# Autodesk Inventor assembly: КВ33.044.500 - Каретка оси Y
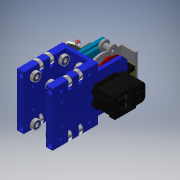
[picture p0: Inventor's stored thumbnail of the model, 180x180]
Saved by Autodesk Inventor 2019 (Build 230136000, 136)
## iProperties
Created: 2019-07-21
Part Number: КВ33.044.500 - Каретка оси Y
Material: Типовые
Document SubType Name: Assembly
Designer: Петров Иван
Mass: 285.838 g
Surface Area: 1117.75 cm^2
Volume: 225.546 cm^3
Density: 1.26732 g/cm^3
Author: Петров Иван
## Documents named in this file (14)
- E:\IVAN\Kvantoriada20192\optimal_gripper\hardware\КВ33.044.700 - Каретка оси Y.iam
- E:\IVAN\Kvantoriada20192\optimal_gripper\hardware\КВ33.044.701 - Щека каретка оси Y.ipt
- C:\Users\Петров Иван\Music\Desktop\palletaizer\Стандартные изделия\Подшипник 624Z.ipt
- E:\IVAN\Kvantoriada20192\optimal_gripper\hardware\Стандартные изделия\Датчик оптический стандартный.ipt
- E:\IVAN\Kvantoriada20192\optimal_gripper\hardware\КВ33.044.702 - Стойка натягивающих роликов оси Y.ipt
- E:\IVAN\Kvantoriada20192\optimal_gripper\hardware\Стандартные изделия\Сервомотор Dynamixel AX-12A\AX-12.iam
- E:\IVAN\Kvantoriada20192\optimal_gripper\hardware\Стандартные изделия\Колесо оптического датчика.ipt
- E:\IVAN\Kvantoriada20192\optimal_gripper\hardware\Стандартные изделия\Шкив большой Makeblock.ipt
- E:\IVAN\Kvantoriada20192\optimal_gripper\hardware\Стандартные изделия\Боковина шкива.ipt
- E:\IVAN\Kvantoriada20192\optimal_gripper\hardware\Стандартные изделия\Шкив плоский Makeblock сборка.iam
- E:\IVAN\Kvantoriada20192\optimal_gripper\hardware\Стандартные изделия\Концевик механический.ipt
- E:\IVAN\Kvantoriada20192\optimal_gripper\hardware\Стандартные изделия\Проставка 5.5 мм.ipt
- E:\IVAN\Kvantoriada20192\optimal_gripper\hardware\КВ33.044.703 - Стойка оптического датчика оси Y.ipt
- E:\IVAN\Kvantoriada20192\optimal_gripper\hardware\КВ33.044.704 - Панель установки принимающей платы оси Y.ipt
## Components (30 placed, 13 different names)
1. КВ33.044.701 - Щека каретка оси Y:1 — Совмещение:1, Совмещение:2, Совмещение:3, Совмещение:4, Совмещение:5, Совмещение:6, 2.5, Совмещение:8, Совмещение:9, Совмещение:10, Совмещение:11, Совмещение:12, Совмещение:13, Совмещение:14, Совмещение:15, Совмещение:16, Совмещение:23, Совмещение:24, Совмещение:25, Совмещение:26, Совмещение:27, Совмещение:28, Совмещение:29, Совмещение:30, Совмещение:31, Совмещение:32, Совмещение:33, Совмещение:34, Совмещение:35, Совмещение:36, Совмещение:37, Совмещение:38, Совмещение:63, Совмещение:66, Совмещение:82, Совмещение:83, Совмещение:84, Совмещение:85, Совмещение:86, Совмещение:87, Совмещение:88, Совмещение:89, Совмещение:94, Совмещение:95, Совмещение:98, Совмещение:99, Совмещение:100
2. Подшипник 624Z:1 — Совмещение:1, Совмещение:8
3. Подшипник 624Z:2 — Совмещение:4, Совмещение:5
4. Подшипник 624Z:3 — Совмещение:3, Совмещение:6
5. Подшипник 624Z:4 — Совмещение:2, 2.5
6. Подшипник 624Z:5 — Совмещение:9, Совмещение:15
7. Подшипник 624Z:6 — Совмещение:10, Совмещение:16
8. Подшипник 624Z:7 — Совмещение:11, Совмещение:13
9. Подшипник 624Z:8 — Совмещение:12, Совмещение:14
10. Подшипник 624Z:9 — Совмещение:23, Совмещение:24
11. Подшипник 624Z:10 — Совмещение:25, Совмещение:26
12. Подшипник 624Z:11 — Совмещение:27, Совмещение:28
13. Подшипник 624Z:12 — Совмещение:29, Совмещение:30
14. Подшипник 624Z:13 — Совмещение:31, Совмещение:32
15. Подшипник 624Z:14 — Совмещение:33, Совмещение:34
16. Подшипник 624Z:15 — Совмещение:35, Совмещение:36
17. Подшипник 624Z:16 — Совмещение:37, Совмещение:38
18. КВ33.044.702 - Стойка натягивающих роликов оси Y:1 — Совмещение:63, Совмещение:80, Касательность:1, Совмещение:81, Касательность:2, Совмещение:82, Совмещение:83, Совмещение:90, Совмещение:101, Совмещение:102
19. AX-12:1 [sub-assembly] — Совмещение:66, Совмещение:94, Совмещение:95, Совмещение:96, Совмещение:97
20. Колесо оптического датчика:1 — Совмещение:71, Совмещение:72, Совмещение:73, Совмещение:74, Совмещение:75, Совмещение:76
21. Проставка 5.5 мм:1 — Совмещение:71, Совмещение:72, Совмещение:73, Совмещение:96, Совмещение:97
22. Шкив большой Makeblock:1 — Совмещение:74, Совмещение:75, Совмещение:76, Совмещение:77, Совмещение:78, Совмещение:79
23. Боковина шкива:1 — Совмещение:77, Совмещение:78, Совмещение:79
24. Шкив плоский Makeblock сборка:1 [sub-assembly] — Совмещение:80, Касательность:1
25. Шкив плоский Makeblock сборка:2 [sub-assembly] — Совмещение:81, Касательность:2
26. Концевик механический:1 — Совмещение:84, Совмещение:85, Совмещение:86
27. Концевик механический:2 — Совмещение:87, Совмещение:88, Совмещение:89
28. КВ33.044.703 - Стойка оптического датчика оси Y:1 — Совмещение:90, Совмещение:93, Заподлицо:1, Заподлицо:2, Совмещение:101, Совмещение:102
29. Датчик оптический стандартный:2 — Совмещение:93, Заподлицо:1, Заподлицо:2
30. КВ33.044.704 - Панель установки принимающей платы оси Y:1 — Совмещение:98, Совмещение:99, Совмещение:100
## Relationships (68: Mate 64, Tangent 2, Flush 2)
- Совмещение:1 [Mate]: КВ33.044.701 - Щека каретка оси Y:1 ↔ Подшипник 624Z:1
- Совмещение:2 [Mate]: КВ33.044.701 - Щека каретка оси Y:1 ↔ Подшипник 624Z:4
- Совмещение:3 [Mate]: КВ33.044.701 - Щека каретка оси Y:1 ↔ Подшипник 624Z:3
- Совмещение:4 [Mate]: КВ33.044.701 - Щека каретка оси Y:1 ↔ Подшипник 624Z:2
- Совмещение:5 [Mate] (2.5 mm): КВ33.044.701 - Щека каретка оси Y:1 ↔ Подшипник 624Z:2
- Совмещение:6 [Mate] (2.5 mm): КВ33.044.701 - Щека каретка оси Y:1 ↔ Подшипник 624Z:3
- 2.5 [Mate] (2.5 mm): КВ33.044.701 - Щека каретка оси Y:1 ↔ Подшипник 624Z:4
- Совмещение:8 [Mate] (2.5 mm): КВ33.044.701 - Щека каретка оси Y:1 ↔ Подшипник 624Z:1
- Совмещение:9 [Mate]: КВ33.044.701 - Щека каретка оси Y:1 ↔ Подшипник 624Z:5
- Совмещение:10 [Mate]: КВ33.044.701 - Щека каретка оси Y:1 ↔ Подшипник 624Z:6
- Совмещение:11 [Mate]: КВ33.044.701 - Щека каретка оси Y:1 ↔ Подшипник 624Z:7
- Совмещение:12 [Mate]: КВ33.044.701 - Щека каретка оси Y:1 ↔ Подшипник 624Z:8
- Совмещение:13 [Mate] (0.5 mm): КВ33.044.701 - Щека каретка оси Y:1 ↔ Подшипник 624Z:7
- Совмещение:14 [Mate] (0.5 mm): КВ33.044.701 - Щека каретка оси Y:1 ↔ Подшипник 624Z:8
- Совмещение:15 [Mate] (0.5 mm): КВ33.044.701 - Щека каретка оси Y:1 ↔ Подшипник 624Z:5
- Совмещение:16 [Mate] (0.5 mm): КВ33.044.701 - Щека каретка оси Y:1 ↔ Подшипник 624Z:6
- Совмещение:23 [Mate]: КВ33.044.701 - Щека каретка оси Y:1 ↔ Подшипник 624Z:9
- Совмещение:24 [Mate] (0.5 mm): КВ33.044.701 - Щека каретка оси Y:1 ↔ Подшипник 624Z:9
- Совмещение:25 [Mate]: КВ33.044.701 - Щека каретка оси Y:1 ↔ Подшипник 624Z:10
- Совмещение:26 [Mate] (0.5 mm): КВ33.044.701 - Щека каретка оси Y:1 ↔ Подшипник 624Z:10
- Совмещение:27 [Mate]: КВ33.044.701 - Щека каретка оси Y:1 ↔ Подшипник 624Z:11
- Совмещение:28 [Mate] (0.5 mm): КВ33.044.701 - Щека каретка оси Y:1 ↔ Подшипник 624Z:11
- Совмещение:29 [Mate]: КВ33.044.701 - Щека каретка оси Y:1 ↔ Подшипник 624Z:12
- Совмещение:30 [Mate] (0.5 mm): КВ33.044.701 - Щека каретка оси Y:1 ↔ Подшипник 624Z:12
- Совмещение:31 [Mate]: КВ33.044.701 - Щека каретка оси Y:1 ↔ Подшипник 624Z:13
- Совмещение:32 [Mate] (2.5 mm): КВ33.044.701 - Щека каретка оси Y:1 ↔ Подшипник 624Z:13
- Совмещение:33 [Mate]: КВ33.044.701 - Щека каретка оси Y:1 ↔ Подшипник 624Z:14
- Совмещение:34 [Mate] (2.5 mm): КВ33.044.701 - Щека каретка оси Y:1 ↔ Подшипник 624Z:14
- Совмещение:35 [Mate] (2.5 mm): КВ33.044.701 - Щека каретка оси Y:1 ↔ Подшипник 624Z:15
- Совмещение:36 [Mate]: КВ33.044.701 - Щека каретка оси Y:1 ↔ Подшипник 624Z:15
- Совмещение:37 [Mate] (2.5 mm): КВ33.044.701 - Щека каретка оси Y:1 ↔ Подшипник 624Z:16
- Совмещение:38 [Mate]: КВ33.044.701 - Щека каретка оси Y:1 ↔ Подшипник 624Z:16
- Совмещение:63 [Mate]: КВ33.044.701 - Щека каретка оси Y:1 ↔ КВ33.044.702 - Стойка натягивающих роликов оси Y:1
- Совмещение:66 [Mate]: КВ33.044.701 - Щека каретка оси Y:1 ↔ AX-12:1
- Совмещение:71 [Mate]: Колесо оптического датчика:1 ↔ Проставка 5.5 мм:1
- Совмещение:72 [Mate]: Колесо оптического датчика:1 ↔ Проставка 5.5 мм:1
- Совмещение:73 [Mate]: Колесо оптического датчика:1 ↔ Проставка 5.5 мм:1
- Совмещение:74 [Mate]: Колесо оптического датчика:1 ↔ Шкив большой Makeblock:1
- Совмещение:75 [Mate]: Колесо оптического датчика:1 ↔ Шкив большой Makeblock:1
- Совмещение:76 [Mate]: Колесо оптического датчика:1 ↔ Шкив большой Makeblock:1
- Совмещение:77 [Mate]: Шкив большой Makeblock:1 ↔ Боковина шкива:1
- Совмещение:78 [Mate]: Шкив большой Makeblock:1 ↔ Боковина шкива:1
- Совмещение:79 [Mate]: Шкив большой Makeblock:1 ↔ Боковина шкива:1
- Совмещение:80 [Mate]: КВ33.044.702 - Стойка натягивающих роликов оси Y:1 ↔ Шкив плоский Makeblock сборка:1
- Касательность:1 [Tangent]: КВ33.044.702 - Стойка натягивающих роликов оси Y:1 ↔ Шкив плоский Makeblock сборка:1
- Совмещение:81 [Mate]: КВ33.044.702 - Стойка натягивающих роликов оси Y:1 ↔ Шкив плоский Makeblock сборка:2
- Касательность:2 [Tangent]: КВ33.044.702 - Стойка натягивающих роликов оси Y:1 ↔ Шкив плоский Makeblock сборка:2
- Совмещение:82 [Mate]: КВ33.044.701 - Щека каретка оси Y:1 ↔ КВ33.044.702 - Стойка натягивающих роликов оси Y:1
- Совмещение:83 [Mate]: КВ33.044.701 - Щека каретка оси Y:1 ↔ КВ33.044.702 - Стойка натягивающих роликов оси Y:1
- Совмещение:84 [Mate]: КВ33.044.701 - Щека каретка оси Y:1 ↔ Концевик механический:1
- Совмещение:85 [Mate]: КВ33.044.701 - Щека каретка оси Y:1 ↔ Концевик механический:1
- Совмещение:86 [Mate]: КВ33.044.701 - Щека каретка оси Y:1 ↔ Концевик механический:1
- Совмещение:87 [Mate]: КВ33.044.701 - Щека каретка оси Y:1 ↔ Концевик механический:2
- Совмещение:88 [Mate]: КВ33.044.701 - Щека каретка оси Y:1 ↔ Концевик механический:2
- Совмещение:89 [Mate]: КВ33.044.701 - Щека каретка оси Y:1 ↔ Концевик механический:2
- Совмещение:90 [Mate]: КВ33.044.702 - Стойка натягивающих роликов оси Y:1 ↔ КВ33.044.703 - Стойка оптического датчика оси Y:1
- Совмещение:93 [Mate]: КВ33.044.703 - Стойка оптического датчика оси Y:1 ↔ Датчик оптический стандартный:2
- Заподлицо:1 [Flush] (-1 mm): КВ33.044.703 - Стойка оптического датчика оси Y:1 ↔ Датчик оптический стандартный:2
- Заподлицо:2 [Flush] (6 mm): КВ33.044.703 - Стойка оптического датчика оси Y:1 ↔ Датчик оптический стандартный:2
- Совмещение:94 [Mate]: КВ33.044.701 - Щека каретка оси Y:1 ↔ AX-12:1
- Совмещение:95 [Mate]: КВ33.044.701 - Щека каретка оси Y:1 ↔ AX-12:1
- Совмещение:96 [Mate]: AX-12:1 ↔ Проставка 5.5 мм:1
- Совмещение:97 [Mate]: AX-12:1 ↔ Проставка 5.5 мм:1
- Совмещение:98 [Mate]: КВ33.044.701 - Щека каретка оси Y:1 ↔ КВ33.044.704 - Панель установки принимающей платы оси Y:1
- Совмещение:99 [Mate]: КВ33.044.701 - Щека каретка оси Y:1 ↔ КВ33.044.704 - Панель установки принимающей платы оси Y:1
- Совмещение:100 [Mate]: КВ33.044.701 - Щека каретка оси Y:1 ↔ КВ33.044.704 - Панель установки принимающей платы оси Y:1
- Совмещение:101 [Mate]: КВ33.044.702 - Стойка натягивающих роликов оси Y:1 ↔ КВ33.044.703 - Стойка оптического датчика оси Y:1
- Совмещение:102 [Mate]: КВ33.044.702 - Стойка натягивающих роликов оси Y:1 ↔ КВ33.044.703 - Стойка оптического датчика оси Y:1
